# Autodesk Inventor assembly: Ensamblaje
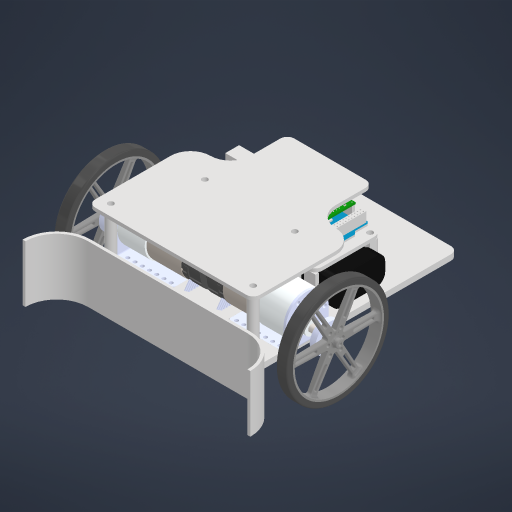
[picture p0: Inventor's stored thumbnail of the model, 512x512]
Saved by Autodesk Inventor 2023 (Build 270158000, 158)
## iProperties
Created: 2022-08-21
Part Number: Ensamblaje
Document SubType Name: Assembly
Designer: marat
Author: marat
## Documents named in this file (19)
- C:\Users\marat\Documents\IRB2001\Parte 1\Ensamblaje.iam
- C:\Users\marat\Documents\IRB2001\Parte 1\Piezas 3D Robot\chasis.ipt
- C:\Users\marat\Documents\IRB2001\Parte 1\Piezas 3D Robot\Bateria.ipt
- C:\Users\marat\Documents\IRB2001\Parte 1\Piezas 3D Robot\pololu-stamped-aluminum-l-bracket-for-37d-mm-metal-gearmotors.ipt
- C:\Users\marat\Documents\IRB2001\Parte 1\Piezas 3D Robot\37d-gearmotor-50-70-encoder.ipt
- C:\Users\marat\Documents\IRB2001\Parte 1\Piezas 3D Robot\pololu-wheel-90x10mm-black.ipt
- C:\Users\marat\Documents\IRB2001\Parte 1\Piezas 3D Robot\pololu-universal-aluminum-mounting-hub-for-6mm-shaft-4-40-holes.ipt
- C:\Users\marat\Documents\IRB2001\Parte 1\Piezas 3D Robot\pololu-stamped-aluminum-l-bracket-for-37d-mm-metal-gearmotors_MIR.ipt
- C:\Users\marat\Documents\IRB2001\Parte 1\Piezas 3D Robot\37d-gearmotor-50-70-encoder_MIR1.ipt
- C:\Users\marat\Documents\IRB2001\Parte 1\Piezas 3D Robot\pololu-wheel-90x10mm-black_MIR.ipt
- C:\Users\marat\Documents\IRB2001\Parte 1\Piezas 3D Robot\pololu-universal-aluminum-mounting-hub-for-6mm-shaft-4-40-holes_MIR.ipt
- C:\Users\marat\Documents\IRB2001\Parte 1\Piezas 3D Robot\pilar.ipt
- C:\Users\marat\Documents\IRB2001\Parte 1\Piezas 3D Robot\chasis_arriba.ipt
- C:\Users\marat\Documents\IRB2001\Parte 1\Piezas 3D Robot\ArduinoMega_STEP_AP203.ipt
- C:\Users\marat\Documents\IRB2001\Parte 1\Piezas 3D Robot\pololu-dual-vnh5019-motor-driver-shield.ipt
- C:\Users\marat\Documents\IRB2001\Parte 1\Piezas 3D Robot\Rueda trasera.ipt
- C:\Users\marat\Documents\IRB2001\Parte 1\Piezas 3D Robot\placa_arduino.ipt
- C:\Users\marat\Documents\IRB2001\Parte 1\Piezas 3D Robot\ancla.ipt
- C:\Users\marat\Documents\IRB2001\Parte 1\Piezas 3D Robot\Pala.ipt
## Components (21 placed, 18 different names)
1. chasis:1 — Mate:24, Mate:25, Mate:26, Mate:27, Mate:29, Mate:30, Mate:32, Mate:34, Mate:36, Mate:40, Mate:49, Mate:51, Flush:6, Mate:53, Mate:55, Mate:56, Mate:58, Mate:59, Mate:60, Angle:1, Angle:2, Flush:12
2. Bateria:1 — Mate:29, Mate:30, Flush:12
3. pololu-stamped-aluminum-l-bracket-for-37d-mm-metal-gearmotors:1 — Mate:1, Mate:6, Mate:27
4. 37d-gearmotor-50-70-encoder:2 — Mate:1, Mate:3, Flush:1, Mate:6, Flush:4, Flush:5
5. pololu-wheel-90x10mm-black:1 — Mate:5, Mate:7, Mate:8
6. pololu-universal-aluminum-mounting-hub-for-6mm-shaft-4-40-holes:2 — Mate:3, Flush:1, Mate:5, Mate:7, Mate:8
7. pololu-stamped-aluminum-l-bracket-for-37d-mm-metal-gearmotors_MIR:1 — Mate:15, Mate:16, Mate:24, Mate:25, Mate:26
8. 37d-gearmotor-50-70-encoder_MIR1:1 — Mate:15, Mate:16, Flush:3, Mate:20, Flush:4, Flush:5
9. pololu-wheel-90x10mm-black_MIR:1 — Mate:17, Mate:18, Mate:19
10. pololu-universal-aluminum-mounting-hub-for-6mm-shaft-4-40-holes_MIR:1 — Mate:17, Mate:18, Mate:19, Flush:3, Mate:20
11. pilar:1 — Mate:36, Mate:37, Angle:1
12. pilar:2 — Mate:32, Mate:62
13. pilar:4 — Mate:34, Mate:63
14. pilar:5 — Mate:40, Mate:61, Angle:2
15. chasis_arriba:1 — Mate:37, Mate:61, Mate:62, Mate:63
16. ArduinoMega_STEP_AP203:1 — Mate:41, Mate:50, Mate:52, Flush:7, Flush:8
17. pololu-dual-vnh5019-motor-driver-shield:1 — Mate:41, Flush:7, Flush:8
18. Rueda trasera:1 — Mate:54, Flush:10, Flush:11
19. placa_arduino:1 — Mate:49, Mate:50, Mate:51, Mate:52, Flush:6
20. ancla:1 — Mate:53, Mate:54, Flush:10, Flush:11, Mate:55, Mate:56
21. Pala:1 — Mate:58, Mate:59, Mate:60
## Relationships (50: Mate 38, Flush 10, Angle 2)
- Mate:1: pololu-stamped-aluminum-l-bracket-for-37d-mm-metal-gearmotors:1 ↔ 37d-gearmotor-50-70-encoder:2
- Mate:3: 37d-gearmotor-50-70-encoder:2 ↔ pololu-universal-aluminum-mounting-hub-for-6mm-shaft-4-40-holes:2
- Flush:1: 37d-gearmotor-50-70-encoder:2 ↔ pololu-universal-aluminum-mounting-hub-for-6mm-shaft-4-40-holes:2
- Mate:5: pololu-wheel-90x10mm-black:1 ↔ pololu-universal-aluminum-mounting-hub-for-6mm-shaft-4-40-holes:2
- Mate:6: pololu-stamped-aluminum-l-bracket-for-37d-mm-metal-gearmotors:1 ↔ 37d-gearmotor-50-70-encoder:2
- Mate:7: pololu-wheel-90x10mm-black:1 ↔ pololu-universal-aluminum-mounting-hub-for-6mm-shaft-4-40-holes:2
- Mate:8: pololu-wheel-90x10mm-black:1 ↔ pololu-universal-aluminum-mounting-hub-for-6mm-shaft-4-40-holes:2
- Mate:15: pololu-stamped-aluminum-l-bracket-for-37d-mm-metal-gearmotors_MIR:1 ↔ 37d-gearmotor-50-70-encoder_MIR1:1
- Mate:16: pololu-stamped-aluminum-l-bracket-for-37d-mm-metal-gearmotors_MIR:1 ↔ 37d-gearmotor-50-70-encoder_MIR1:1
- Mate:17: pololu-wheel-90x10mm-black_MIR:1 ↔ pololu-universal-aluminum-mounting-hub-for-6mm-shaft-4-40-holes_MIR:1
- Mate:18: pololu-wheel-90x10mm-black_MIR:1 ↔ pololu-universal-aluminum-mounting-hub-for-6mm-shaft-4-40-holes_MIR:1
- Mate:19: pololu-wheel-90x10mm-black_MIR:1 ↔ pololu-universal-aluminum-mounting-hub-for-6mm-shaft-4-40-holes_MIR:1
- Flush:3: 37d-gearmotor-50-70-encoder_MIR1:1 ↔ pololu-universal-aluminum-mounting-hub-for-6mm-shaft-4-40-holes_MIR:1
- Mate:20: 37d-gearmotor-50-70-encoder_MIR1:1 ↔ pololu-universal-aluminum-mounting-hub-for-6mm-shaft-4-40-holes_MIR:1
- Flush:4: 37d-gearmotor-50-70-encoder:2 ↔ 37d-gearmotor-50-70-encoder_MIR1:1
- Flush:5: 37d-gearmotor-50-70-encoder:2 ↔ 37d-gearmotor-50-70-encoder_MIR1:1
- Mate:24: chasis:1 ↔ pololu-stamped-aluminum-l-bracket-for-37d-mm-metal-gearmotors_MIR:1
- Mate:25: chasis:1 ↔ pololu-stamped-aluminum-l-bracket-for-37d-mm-metal-gearmotors_MIR:1
- Mate:26: chasis:1 ↔ pololu-stamped-aluminum-l-bracket-for-37d-mm-metal-gearmotors_MIR:1
- Mate:27: chasis:1 ↔ pololu-stamped-aluminum-l-bracket-for-37d-mm-metal-gearmotors:1
- Mate:29: chasis:1 ↔ Bateria:1
- Mate:30: chasis:1 ↔ Bateria:1
- Mate:32: chasis:1 ↔ pilar:2
- Mate:34: chasis:1 ↔ pilar:4
- Mate:36: chasis:1 ↔ pilar:1
- Mate:37: pilar:1 ↔ chasis_arriba:1
- Mate:40: chasis:1 ↔ pilar:5
- Mate:41: ArduinoMega_STEP_AP203:1 ↔ pololu-dual-vnh5019-motor-driver-shield:1
- Mate:49: chasis:1 ↔ placa_arduino:1
- Mate:50: ArduinoMega_STEP_AP203:1 ↔ placa_arduino:1
- Mate:51: chasis:1 ↔ placa_arduino:1
- Mate:52: ArduinoMega_STEP_AP203:1 ↔ placa_arduino:1
- Flush:6: chasis:1 ↔ placa_arduino:1
- Flush:7: ArduinoMega_STEP_AP203:1 ↔ pololu-dual-vnh5019-motor-driver-shield:1
- Flush:8: ArduinoMega_STEP_AP203:1 ↔ pololu-dual-vnh5019-motor-driver-shield:1
- Mate:53: chasis:1 ↔ ancla:1
- Mate:54: Rueda trasera:1 ↔ ancla:1
- Flush:10 (2.5 mm): Rueda trasera:1 ↔ ancla:1
- Flush:11 (-3 mm): Rueda trasera:1 ↔ ancla:1
- Mate:55: chasis:1 ↔ ancla:1
- Mate:56: chasis:1 ↔ ancla:1
- Mate:58: chasis:1 ↔ Pala:1
- Mate:59: chasis:1 ↔ Pala:1
- Mate:60: chasis:1 ↔ Pala:1
- Mate:61: pilar:5 ↔ chasis_arriba:1
- Mate:62: pilar:2 ↔ chasis_arriba:1
- Mate:63: pilar:4 ↔ chasis_arriba:1
- Angle:1 (0 deg): chasis:1 ↔ pilar:1
- Angle:2 (0 deg): chasis:1 ↔ pilar:5
- Flush:12 (7.399 mm): chasis:1 ↔ Bateria:1
